# Autodesk Inventor assembly: PART NUMBER
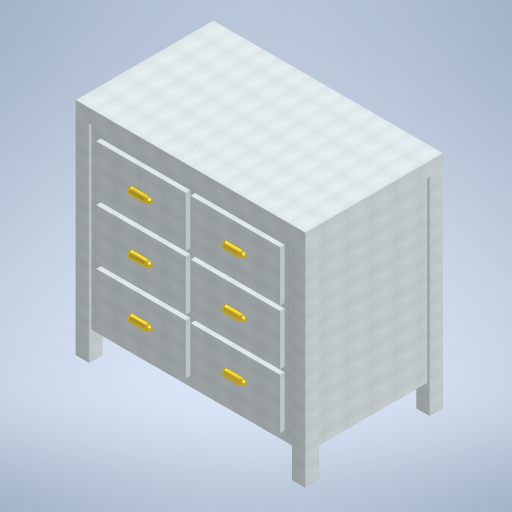
[picture p0: Inventor's stored thumbnail of the model, 512x512]
Saved by Autodesk Inventor 2023 (Build 270158000, 158)
## iProperties
Company: Jay's Dressers
RuleStatus: InUse
Created: 2021-10-04
Document SubType Name: Assembly
Designer: Admin
Part Number: PART NUMBER
Author: Admin
Title: Dresser Assembly
## Documents named in this file (4)
- C:\Users\Admin\source\repos\CadflairWebApplication\Inventor Files\Jays Dressers\Dresser Assembly\Dresser Assembly.iam
- C:\Users\Admin\source\repos\CadflairWebApplication\Inventor Files\Jays Dressers\Dresser Assembly\Dresser Frame.iam
- C:\Users\Admin\source\repos\CadflairWebApplication\Inventor Files\Jays Dressers\Dresser Assembly\Drawer\Drawer Assembly.iam
- C:\Users\Admin\source\repos\CadflairWebApplication\Inventor Files\Jays Dressers\Dresser Assembly\Dresser SKELETON.ipt
## Components (7 placed, 2 different names)
1. Dresser Frame:1 [sub-assembly] — Mate:1, Mate:2, Mate:3
2. Drawer Assembly:1 [sub-assembly] — Mate:1, Mate:2, Mate:3
3. Drawer Assembly:2 [sub-assembly]
4. Drawer Assembly:3 [sub-assembly]
5. Drawer Assembly:4 [sub-assembly]
6. Drawer Assembly:5 [sub-assembly]
7. Drawer Assembly:6 [sub-assembly]
## Component patterns: Drawer Pattern (6 elements)
## Relationships (3: Mate 3)
- Mate:1: Dresser Frame:1 ↔ Drawer Assembly:1
- Mate:2: Dresser Frame:1 ↔ Drawer Assembly:1
- Mate:3 (6.35 mm): Dresser Frame:1 ↔ Drawer Assembly:1
## Named parameters: drawerHeight = 228.6 mm, drawerVerticalOffset = 76.2 mm, drawerWidth = 444.5 mm, drawerHorizontalOffset = 76.2 mm, drawerRows = 3, drawerColumns = 2, rowSpacing = 304.8 mm, columnSpacing = 520.7 mm, rows = 3, columns = 2
